# Autodesk Inventor assembly: daVinciHead_FrameWork
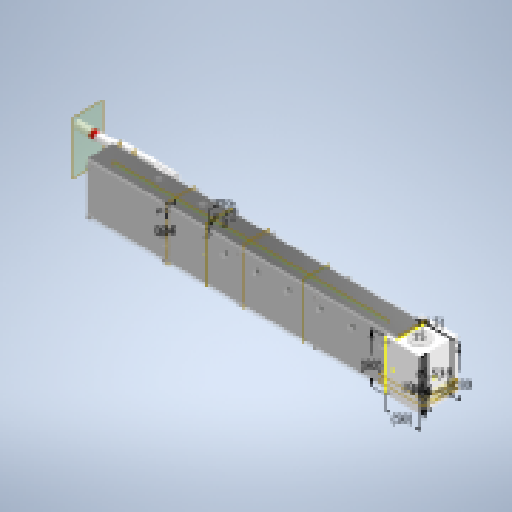
[picture p0: Inventor's stored thumbnail of the model, 512x512]
Saved by Autodesk Inventor 2024 (Build 280153000, 153)
## iProperties
Created: 2022-05-05
Part Number: daVinciHead_FrameWork
Document SubType Name: Assembly
Designer: 123St
Mass: 798.994 g
Surface Area: 3107.96 cm^2
Volume: 766.703 cm^3
Author: 123St
## Documents named in this file (14)
- C:\Users\AEWALDER\Documents\Inventor\03_CurrentProjects\MasterThesis\PSM_V1_Rillenkugellager\Ueberarbeiteter DaVincikopf\daVinciHead_FrameWork.iam
- C:\Users\AEWALDER\Documents\Inventor\03_CurrentProjects\MasterThesis\PSM_V1_Rillenkugellager\Ueberarbeiteter DaVincikopf\Fuehrungsschiene.ipt
- C:\Users\AEWALDER\Documents\Inventor\03_CurrentProjects\MasterThesis\PSM_V1_Rillenkugellager\Ueberarbeiteter DaVincikopf\Zahnradbahn.ipt
- C:\Users\AEWALDER\Documents\Inventor\03_CurrentProjects\MasterThesis\PSM_V1_Rillenkugellager\Back plate profile.ipt
- C:\Users\AEWALDER\Documents\Inventor\03_CurrentProjects\MasterThesis\PSM_V1_Rillenkugellager\Slot profile.ipt
- C:\Users\AEWALDER\Documents\Inventor\03_CurrentProjects\MasterThesis\PSM_V1_Rillenkugellager\Guide.ipt
- C:\Users\AEWALDER\Documents\Inventor\03_CurrentProjects\MasterThesis\PSM_V1_Rillenkugellager\ContentCenter\de-DE\ISO 4762(2)\ISO 4762 - M3 x 10ISO.ipt
- C:\Users\AEWALDER\Documents\Inventor\03_CurrentProjects\MasterThesis\PSM_V1_Rillenkugellager\ContentCenter\de-DE\ISO 4762(2)\ISO 4762 - M3 x 12ISO.ipt
- C:\Users\AEWALDER\Documents\Inventor\03_CurrentProjects\MasterThesis\PSM_V1_Rillenkugellager\ContentCenter\de-DE\ISO 10642(1)\ISO 10642 - M3 x  8.ipt
- C:\Users\AEWALDER\Documents\Inventor\03_CurrentProjects\MasterThesis\PSM_V1_Rillenkugellager\ContentCenter\de-DE\ISO 4762(2)\ISO 4762 - M3 x 16ISO.ipt
- C:\Users\AEWALDER\Documents\Inventor\03_CurrentProjects\MasterThesis\PSM_V1_Rillenkugellager\Sensor_Box_Assembly.ipt.iam
- C:\Users\AEWALDER\Documents\Inventor\03_CurrentProjects\MasterThesis\PSM_V1_Rillenkugellager\ContentCenter\de-DE\ISO 4762(2)\ISO 4762 - M3 x 20ISO.ipt
- C:\Users\AEWALDER\Documents\Inventor\03_CurrentProjects\MasterThesis\PSM_V1_Rillenkugellager\Tension_Thingy_v2.iam
- Sensor_Box_Assembly.ipt
## Components (37 placed, 12 different names)
1. Fuehrungsschiene:1 — Passend:40, Passend:51, Passend:53, Passend:55, Passend:57, Passend:59, Passend:61, Passend:63, Passend:65, Passend:71, Passend:73, Passend:77, Passend:81, Passend:83, Passend:87, Passend:101, Passend:105, Passend:106, Passend:112, Passend:115, Passend:116, Passend:117, Passend:118, Passend:119, Passend:120, Passend:123, Fluchtend:1, Passend:124, Passend:125, Passend:137, Passend:139, Mate:161, Mate:162
2. Back plate profile:1 — Passend:52, Passend:54, Passend:56, Passend:58, Passend:60, Passend:62, Passend:64, Passend:66, Passend:101, Passend:111, Passend:136
3. Slot profile:1 — Passend:40, Passend:43, Passend:72, Passend:74, Passend:78, Passend:82, Passend:84, Passend:88, Passend:112, Passend:121, Passend:122, Passend:138
4. Guide:1 — Passend:43, Passend:121, Passend:122, Passend:126, Passend:127, Passend:128, Passend:129, Passend:130, Passend:131, Passend:132, Passend:133
5. Zahnradbahn:1 — Passend:123, Fluchtend:1, Passend:124, Passend:125
6. ISO 4762 M3 x 10:2 — Passend:51, Passend:52
7. ISO 4762 M3 x 10:3 — Passend:53, Passend:54
8. ISO 4762 M3 x 10:4 — Passend:55, Passend:56
9. ISO 4762 M3 x 10:5 — Passend:57, Passend:58
10. ISO 4762 M3 x 10:6 — Passend:59, Passend:60
11. ISO 4762 M3 x 10:7 — Passend:61, Passend:62
12. ISO 4762 M3 x 10:8 — Passend:63, Passend:64, Passend:111
13. ISO 4762 M3 x 10:9 — Passend:65, Passend:66
14. ISO 4762 M3 x 12:2 — Passend:71, Passend:72
15. ISO 4762 M3 x 12:3 — Passend:73, Passend:74
16. ISO 4762 M3 x 12:5 — Passend:77, Passend:78
17. ISO 4762 M3 x 12:7 — Passend:81, Passend:82
18. ISO 4762 M3 x 12:8 — Passend:83, Passend:84
19. ISO 4762 M3 x 12:10 — Passend:87, Passend:88
20. ISO 10642 M3x8:1 — Passend:115
21. ISO 10642 M3x8:2 — Passend:116
22. ISO 10642 M3x8:3 — Passend:117
23. ISO 10642 M3x8:4 — Passend:118
24. ISO 10642 M3x8:5 — Passend:119
25. ISO 10642 M3x8:6 — Passend:120
26. ISO 4762 M3 x 16:1 — Passend:126, Passend:127
27. ISO 4762 M3 x 16:2 — Passend:128, Passend:129
28. ISO 4762 M3 x 16:3 — Passend:130, Passend:131
29. ISO 4762 M3 x 16:4 — Passend:132, Passend:133
30. Sensor_Box_Assembly.ipt:1 [sub-assembly] — Passend:136, Passend:137, Passend:138, Passend:140, Passend:141, Passend:142, Passend:143, Passend:144, Passend:145, Passend:146, Passend:147, Passend:148, Passend:149, Passend:150
31. ISO 4762 M3 x 20:1 — Passend:139, Passend:140
32. ISO 4762 M3 x 20:2 — Passend:141, Passend:142
33. ISO 4762 M3 x 20:3 — Passend:143, Passend:144
34. ISO 4762 M3 x 20:4 — Passend:145, Passend:146
35. ISO 4762 M3 x 16:5 — Passend:147, Passend:148
36. ISO 4762 M3 x 16:6 — Passend:149, Passend:150
37. Tension_Thingy_v2:1 [sub-assembly] — Mate:161, Mate:162
## Relationships (72: Mate 71, Flush 1)
- Passend:40 [Mate]: Fuehrungsschiene:1 ↔ Slot profile:1
- Passend:43 [Mate]: Slot profile:1 ↔ Guide:1
- Passend:51 [Mate]: Fuehrungsschiene:1 ↔ ISO 4762 M3 x 10:2
- Passend:52 [Mate]: Back plate profile:1 ↔ ISO 4762 M3 x 10:2
- Passend:53 [Mate]: Fuehrungsschiene:1 ↔ ISO 4762 M3 x 10:3
- Passend:54 [Mate]: Back plate profile:1 ↔ ISO 4762 M3 x 10:3
- Passend:55 [Mate]: Fuehrungsschiene:1 ↔ ISO 4762 M3 x 10:4
- Passend:56 [Mate]: Back plate profile:1 ↔ ISO 4762 M3 x 10:4
- Passend:57 [Mate]: Fuehrungsschiene:1 ↔ ISO 4762 M3 x 10:5
- Passend:58 [Mate]: Back plate profile:1 ↔ ISO 4762 M3 x 10:5
- Passend:59 [Mate]: Fuehrungsschiene:1 ↔ ISO 4762 M3 x 10:6
- Passend:60 [Mate]: Back plate profile:1 ↔ ISO 4762 M3 x 10:6
- Passend:61 [Mate]: Fuehrungsschiene:1 ↔ ISO 4762 M3 x 10:7
- Passend:62 [Mate]: Back plate profile:1 ↔ ISO 4762 M3 x 10:7
- Passend:63 [Mate]: Fuehrungsschiene:1 ↔ ISO 4762 M3 x 10:8
- Passend:64 [Mate]: Back plate profile:1 ↔ ISO 4762 M3 x 10:8
- Passend:65 [Mate]: Fuehrungsschiene:1 ↔ ISO 4762 M3 x 10:9
- Passend:66 [Mate]: Back plate profile:1 ↔ ISO 4762 M3 x 10:9
- Passend:71 [Mate]: Fuehrungsschiene:1 ↔ ISO 4762 M3 x 12:2
- Passend:72 [Mate]: Slot profile:1 ↔ ISO 4762 M3 x 12:2
- Passend:73 [Mate]: Fuehrungsschiene:1 ↔ ISO 4762 M3 x 12:3
- Passend:74 [Mate]: Slot profile:1 ↔ ISO 4762 M3 x 12:3
- Passend:77 [Mate]: Fuehrungsschiene:1 ↔ ISO 4762 M3 x 12:5
- Passend:78 [Mate]: Slot profile:1 ↔ ISO 4762 M3 x 12:5
- Passend:81 [Mate]: Fuehrungsschiene:1 ↔ ISO 4762 M3 x 12:7
- Passend:82 [Mate]: Slot profile:1 ↔ ISO 4762 M3 x 12:7
- Passend:83 [Mate]: Fuehrungsschiene:1 ↔ ISO 4762 M3 x 12:8
- Passend:84 [Mate]: Slot profile:1 ↔ ISO 4762 M3 x 12:8
- Passend:87 [Mate]: Fuehrungsschiene:1 ↔ ISO 4762 M3 x 12:10
- Passend:88 [Mate]: Slot profile:1 ↔ ISO 4762 M3 x 12:10
- Passend:101 [Mate]: Fuehrungsschiene:1 ↔ Back plate profile:1
- Passend:105 [Mate]: Fuehrungsschiene:1
- Passend:106 [Mate]: Fuehrungsschiene:1
- Passend:111 [Mate]: Back plate profile:1 ↔ ISO 4762 M3 x 10:8
- Passend:112 [Mate]: Fuehrungsschiene:1 ↔ Slot profile:1
- Passend:115 [Mate]: Fuehrungsschiene:1 ↔ ISO 10642 M3x8:1
- Passend:116 [Mate]: Fuehrungsschiene:1 ↔ ISO 10642 M3x8:2
- Passend:117 [Mate]: Fuehrungsschiene:1 ↔ ISO 10642 M3x8:3
- Passend:118 [Mate]: Fuehrungsschiene:1 ↔ ISO 10642 M3x8:4
- Passend:119 [Mate]: Fuehrungsschiene:1 ↔ ISO 10642 M3x8:5
- Passend:120 [Mate]: Fuehrungsschiene:1 ↔ ISO 10642 M3x8:6
- Passend:121 [Mate]: Slot profile:1 ↔ Guide:1
- Passend:122 [Mate]: Slot profile:1 ↔ Guide:1
- Passend:123 [Mate]: Fuehrungsschiene:1 ↔ Zahnradbahn:1
- Fluchtend:1 [Flush]: Fuehrungsschiene:1 ↔ Zahnradbahn:1
- Passend:124 [Mate]: Fuehrungsschiene:1 ↔ Zahnradbahn:1
- Passend:125 [Mate]: Fuehrungsschiene:1 ↔ Zahnradbahn:1
- Passend:126 [Mate]: Guide:1 ↔ ISO 4762 M3 x 16:1
- Passend:127 [Mate]: Guide:1 ↔ ISO 4762 M3 x 16:1
- Passend:128 [Mate]: Guide:1 ↔ ISO 4762 M3 x 16:2
- Passend:129 [Mate]: Guide:1 ↔ ISO 4762 M3 x 16:2
- Passend:130 [Mate]: Guide:1 ↔ ISO 4762 M3 x 16:3
- Passend:131 [Mate]: Guide:1 ↔ ISO 4762 M3 x 16:3
- Passend:132 [Mate]: Guide:1 ↔ ISO 4762 M3 x 16:4
- Passend:133 [Mate]: Guide:1 ↔ ISO 4762 M3 x 16:4
- Passend:136 [Mate]: Back plate profile:1 ↔ Sensor_Box_Assembly.ipt:1
- Passend:137 [Mate]: Fuehrungsschiene:1 ↔ Sensor_Box_Assembly.ipt:1
- Passend:138 [Mate]: Slot profile:1 ↔ Sensor_Box_Assembly.ipt:1
- Passend:139 [Mate]: Fuehrungsschiene:1 ↔ ISO 4762 M3 x 20:1
- Passend:140 [Mate]: Sensor_Box_Assembly.ipt:1 ↔ ISO 4762 M3 x 20:1
- Passend:141 [Mate]: Sensor_Box_Assembly.ipt:1 ↔ ISO 4762 M3 x 20:2
- Passend:142 [Mate]: Sensor_Box_Assembly.ipt:1 ↔ ISO 4762 M3 x 20:2
- Passend:143 [Mate]: Sensor_Box_Assembly.ipt:1 ↔ ISO 4762 M3 x 20:3
- Passend:144 [Mate]: Sensor_Box_Assembly.ipt:1 ↔ ISO 4762 M3 x 20:3
- Passend:145 [Mate]: Sensor_Box_Assembly.ipt:1 ↔ ISO 4762 M3 x 20:4
- Passend:146 [Mate]: Sensor_Box_Assembly.ipt:1 ↔ ISO 4762 M3 x 20:4
- Passend:147 [Mate]: Sensor_Box_Assembly.ipt:1 ↔ ISO 4762 M3 x 16:5
- Passend:148 [Mate]: Sensor_Box_Assembly.ipt:1 ↔ ISO 4762 M3 x 16:5
- Passend:149 [Mate]: Sensor_Box_Assembly.ipt:1 ↔ ISO 4762 M3 x 16:6
- Passend:150 [Mate]: Sensor_Box_Assembly.ipt:1 ↔ ISO 4762 M3 x 16:6
- Mate:161: Fuehrungsschiene:1 ↔ Tension_Thingy_v2:1
- Mate:162: Fuehrungsschiene:1 ↔ Tension_Thingy_v2:1
